# Autodesk Inventor assembly: Left Leg
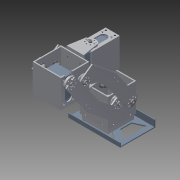
[picture p0: Inventor's stored thumbnail of the model, 180x180]
Saved by Autodesk Inventor 2013 (Build 170138000, 138)
## iProperties
Created: 2014-05-10
Part Number: Left Leg
Document SubType Name: Assembly
Designer: andou
Author: andou
## Documents named in this file (17)
- C:\Users\andou\Documents\Inventor\RoboticsProject\project_4\Robot\Leg\pre Leg.iam
- C:\Users\andou\Documents\Inventor\RoboticsProject\project_4\Robot\All Common\Serial_Case.ipt
- C:\Users\andou\Documents\Inventor\RoboticsProject\project_4\Robot\All Common\Bracket.ipt
- C:\Users\andou\Documents\Inventor\RoboticsProject\project_4\Robot\All Common\KRS-2542HV.ipt
- C:\Users\andou\Documents\Inventor\RoboticsProject\project_4\Robot\All Common\Low_Height_Horn.ipt
- C:\Users\andou\Documents\Inventor\RoboticsProject\project_4\Robot\All Common\Washer(M4).ipt
- C:\Users\andou\Documents\Inventor\RoboticsProject\project_4\Robot\All Common\Nylon_Nat(M4).ipt
- C:\Users\andou\Documents\Inventor\RoboticsProject\project_4\Robot\All Common\Cap(M4-15).ipt
- C:\Users\andou\Documents\Inventor\RoboticsProject\project_4\Robot\Free_Horn\Free_Horn.iam
- C:\Users\andou\Documents\Inventor\RoboticsProject\project_4\Robot\Free_Horn\Low Free Horn.iam
- C:\Users\andou\Documents\Inventor\RoboticsProject\project_4\Robot\All Common\Horn_Spacer.ipt
- C:\Users\andou\Documents\Inventor\RoboticsProject\project_4\Robot\All Common\Cap(M3-6).ipt
- C:\Users\andou\Documents\Inventor\RoboticsProject\project_4\Robot\Leg\Common\Parallel_Case.ipt
- C:\Users\andou\Documents\Inventor\RoboticsProject\project_4\Robot\Leg\Common\Sole_Spacer.ipt
- C:\Users\andou\Documents\Inventor\RoboticsProject\project_4\Robot\Leg\Common\Link_Flame.ipt
- C:\Users\andou\Documents\Inventor\RoboticsProject\project_4\Robot\Leg\Right_Leg\Right_Parallel_Case.ipt
- C:\Users\andou\Documents\Inventor\RoboticsProject\project_4\Robot\Leg\Right_Leg\Right_Sole.ipt
## Components (49 placed, 16 different names)
1. Serial_Case:1 — 挿入:1, 挿入:2, 挿入:4, 挿入:10
2. Bracket:1 — 挿入:8, 挿入:9, 挿入:12, 挿入:13, 挿入:71, 挿入:72
3. KRS-2542HV:1 — 挿入:1, 挿入:2, 挿入:3
4. Low_Height_Horn:1 — 挿入:3, 挿入:8, 挿入:9, 挿入:91
5. Washer(M4):1 — 挿入:4, 挿入:5
6. Nylon_Nat(M4):1 — 挿入:5
7. Cap(M4-15):1 — 挿入:11
8. Low Free Horn:1 [sub-assembly] — 挿入:10, 挿入:11, 挿入:12, 挿入:13
9. KRS-2542HV:2 — 挿入:17, 挿入:73, 挿入:74
10. Horn_Spacer:1 — 挿入:16, 挿入:29, 挿入:75, 挿入:88, 挿入:89, 挿入:90
11. Nylon_Nat(M4):2 — 挿入:22
12. Nylon_Nat(M4):3 — 挿入:21
13. Nylon_Nat(M4):4 — 挿入:20
14. Washer(M4):2 — 挿入:22, 挿入:83
15. Washer(M4):3 — 挿入:21, 挿入:84
16. Washer(M4):4 — 挿入:20, 挿入:85
17. Low_Height_Horn:2 — 挿入:16, 挿入:17, 挿入:89, 挿入:90
18. Free_Horn:1 [sub-assembly] — 挿入:32, 挿入:77, 挿入:79, 挿入:81
19. Free_Horn:2 [sub-assembly] — 挿入:31, 挿入:56, 挿入:57, 挿入:76
20. Free_Horn:3 [sub-assembly] — 挿入:30, 挿入:78, 挿入:80, 挿入:82
21. Cap(M3-6):1 — 挿入:29
22. Cap(M4-15):2 — 挿入:32
23. Cap(M4-15):3 — 挿入:31
24. Cap(M4-15):4 — 挿入:30
25. Parallel_Case:1 — 挿入:37, 挿入:38, 挿入:39, 挿入:40, 挿入:41, 挿入:42, 挿入:43, 挿入:44, 挿入:65, 挿入:66
26. Sole_Spacer:1 — 挿入:65, 挿入:66, 挿入:86, 挿入:87
27. Free_Horn:4 [sub-assembly] — 挿入:44, 挿入:52, 挿入:53, 挿入:67
28. Free_Horn:5 [sub-assembly] — 挿入:43, 挿入:51, 挿入:54, 挿入:68
29. Free_Horn:6 [sub-assembly] — 挿入:42, 挿入:45, 挿入:58, 挿入:59
30. Free_Horn:7 [sub-assembly] — 挿入:41, 挿入:46, 挿入:55, 挿入:60
31. Nylon_Nat(M4):5 — 挿入:33
32. Nylon_Nat(M4):6 — 挿入:34
33. Nylon_Nat(M4):7 — 挿入:35
34. Nylon_Nat(M4):8 — 挿入:36
35. Cap(M4-15):7 — 挿入:46
36. Cap(M4-15):8 — 挿入:45
37. Washer(M4):5 — 挿入:33, 挿入:40
38. Washer(M4):6 — 挿入:34, 挿入:39
39. Washer(M4):7 — 挿入:35, 挿入:38
40. Washer(M4):8 — 挿入:36, 挿入:37
41. Link_Flame:1 — 挿入:52, 挿入:53, 挿入:80, 挿入:82
42. Link_Flame:2 — 挿入:51, 挿入:54, 挿入:79, 挿入:81
43. Link_Flame:3 — 挿入:56, 挿入:57, 挿入:58, 挿入:59
44. Link_Flame:4 — 挿入:55, 挿入:60, 挿入:75, 挿入:88
45. Cap(M4-15):9 — 挿入:67
46. Cap(M4-15):10 — 挿入:68
47. Right_Parallel_Case:1 — 挿入:71, 挿入:72, 挿入:73, 挿入:74, 挿入:76, 挿入:77, 挿入:78, 挿入:83, 挿入:84, 挿入:85
48. Right_Sole:1 — 挿入:86, 挿入:87
49. Cap(M3-6):2 — 挿入:91
## Relationships (69: Insert 69)
- 挿入:1 [Insert]: Serial_Case:1 ↔ KRS-2542HV:1
- 挿入:2 [Insert]: Serial_Case:1 ↔ KRS-2542HV:1
- 挿入:3 [Insert]: KRS-2542HV:1 ↔ Low_Height_Horn:1
- 挿入:4 [Insert]: Serial_Case:1 ↔ Washer(M4):1
- 挿入:5 [Insert]: Washer(M4):1 ↔ Nylon_Nat(M4):1
- 挿入:8 [Insert]: Bracket:1 ↔ Low_Height_Horn:1
- 挿入:9 [Insert]: Bracket:1 ↔ Low_Height_Horn:1
- 挿入:10 [Insert]: Serial_Case:1 ↔ Low Free Horn:1
- 挿入:11 [Insert]: Cap(M4-15):1 ↔ Low Free Horn:1
- 挿入:12 [Insert]: Bracket:1 ↔ Low Free Horn:1
- 挿入:13 [Insert]: Bracket:1 ↔ Low Free Horn:1
- 挿入:16 [Insert]: Horn_Spacer:1 ↔ Low_Height_Horn:2
- 挿入:17 [Insert]: KRS-2542HV:2 ↔ Low_Height_Horn:2
- 挿入:20 [Insert]: Nylon_Nat(M4):4 ↔ Washer(M4):4
- 挿入:21 [Insert]: Nylon_Nat(M4):3 ↔ Washer(M4):3
- 挿入:22 [Insert]: Nylon_Nat(M4):2 ↔ Washer(M4):2
- 挿入:29 [Insert]: Horn_Spacer:1 ↔ Cap(M3-6):1
- 挿入:30 [Insert]: Free_Horn:3 ↔ Cap(M4-15):4
- 挿入:31 [Insert]: Free_Horn:2 ↔ Cap(M4-15):3
- 挿入:32 [Insert]: Free_Horn:1 ↔ Cap(M4-15):2
- 挿入:33 [Insert]: Nylon_Nat(M4):5 ↔ Washer(M4):5
- 挿入:34 [Insert]: Nylon_Nat(M4):6 ↔ Washer(M4):6
- 挿入:35 [Insert]: Nylon_Nat(M4):7 ↔ Washer(M4):7
- 挿入:36 [Insert]: Nylon_Nat(M4):8 ↔ Washer(M4):8
- 挿入:37 [Insert]: Parallel_Case:1 ↔ Washer(M4):8
- 挿入:38 [Insert]: Parallel_Case:1 ↔ Washer(M4):7
- 挿入:39 [Insert]: Parallel_Case:1 ↔ Washer(M4):6
- 挿入:40 [Insert]: Parallel_Case:1 ↔ Washer(M4):5
- 挿入:41 [Insert]: Parallel_Case:1 ↔ Free_Horn:7
- 挿入:42 [Insert]: Parallel_Case:1 ↔ Free_Horn:6
- 挿入:43 [Insert]: Parallel_Case:1 ↔ Free_Horn:5
- 挿入:44 [Insert]: Parallel_Case:1 ↔ Free_Horn:4
- 挿入:45 [Insert]: Free_Horn:6 ↔ Cap(M4-15):8
- 挿入:46 [Insert]: Free_Horn:7 ↔ Cap(M4-15):7
- 挿入:51 [Insert]: Free_Horn:5 ↔ Link_Flame:2
- 挿入:52 [Insert]: Free_Horn:4 ↔ Link_Flame:1
- 挿入:53 [Insert]: Free_Horn:4 ↔ Link_Flame:1
- 挿入:54 [Insert]: Free_Horn:5 ↔ Link_Flame:2
- 挿入:55 [Insert]: Free_Horn:7 ↔ Link_Flame:4
- 挿入:56 [Insert]: Free_Horn:2 ↔ Link_Flame:3
- 挿入:57 [Insert]: Free_Horn:2 ↔ Link_Flame:3
- 挿入:58 [Insert]: Free_Horn:6 ↔ Link_Flame:3
- 挿入:59 [Insert]: Free_Horn:6 ↔ Link_Flame:3
- 挿入:60 [Insert]: Free_Horn:7 ↔ Link_Flame:4
- 挿入:65 [Insert]: Parallel_Case:1 ↔ Sole_Spacer:1
- 挿入:66 [Insert]: Parallel_Case:1 ↔ Sole_Spacer:1
- 挿入:67 [Insert]: Free_Horn:4 ↔ Cap(M4-15):9
- 挿入:68 [Insert]: Free_Horn:5 ↔ Cap(M4-15):10
- 挿入:71 [Insert]: Bracket:1 ↔ Right_Parallel_Case:1
- 挿入:72 [Insert]: Bracket:1 ↔ Right_Parallel_Case:1
- 挿入:73 [Insert]: KRS-2542HV:2 ↔ Right_Parallel_Case:1
- 挿入:74 [Insert]: KRS-2542HV:2 ↔ Right_Parallel_Case:1
- 挿入:75 [Insert]: Horn_Spacer:1 ↔ Link_Flame:4
- 挿入:76 [Insert]: Free_Horn:2 ↔ Right_Parallel_Case:1
- 挿入:77 [Insert]: Free_Horn:1 ↔ Right_Parallel_Case:1
- 挿入:78 [Insert]: Free_Horn:3 ↔ Right_Parallel_Case:1
- 挿入:79 [Insert]: Free_Horn:1 ↔ Link_Flame:2
- 挿入:80 [Insert]: Free_Horn:3 ↔ Link_Flame:1
- 挿入:81 [Insert]: Free_Horn:1 ↔ Link_Flame:2
- 挿入:82 [Insert]: Free_Horn:3 ↔ Link_Flame:1
- 挿入:83 [Insert]: Washer(M4):2 ↔ Right_Parallel_Case:1
- 挿入:84 [Insert]: Washer(M4):3 ↔ Right_Parallel_Case:1
- 挿入:85 [Insert]: Washer(M4):4 ↔ Right_Parallel_Case:1
- 挿入:86 [Insert]: Sole_Spacer:1 ↔ Right_Sole:1
- 挿入:87 [Insert]: Sole_Spacer:1 ↔ Right_Sole:1
- 挿入:88 [Insert]: Horn_Spacer:1 ↔ Link_Flame:4
- 挿入:89 [Insert]: Horn_Spacer:1 ↔ Low_Height_Horn:2
- 挿入:90 [Insert]: Horn_Spacer:1 ↔ Low_Height_Horn:2
- 挿入:91 [Insert]: Low_Height_Horn:1 ↔ Cap(M3-6):2
